# Autodesk Inventor assembly: Plataforma_giratoria_4p
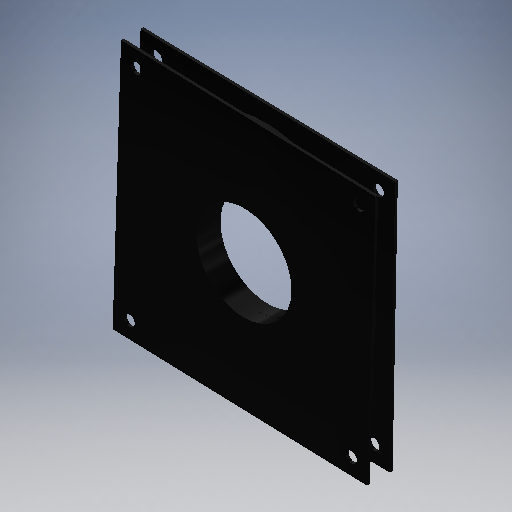
[picture p0: Inventor's stored thumbnail of the model, 512x512]
Saved by Autodesk Inventor 2025.2 (Build 292293000, 293)
## iProperties
Created: 2025-04-27
Part Number: Plataforma_giratoria_4p
Document SubType Name: Assembly
Designer: Tiago
Author: Tiago
## Documents named in this file (2)
- C:\Users\Tiago\Documents\Inventor\Exp. Braço v1\Plataforma_giratoria_4p.iam
- C:\Users\Tiago\Documents\Inventor\Exp. Braço v1\plataforma_giratória_94L)4polegadas).ipt
## Components (2 placed, 1 different names)
1. plataforma_giratória_94L)4polegadas):1 — Mate:1, Mate:2, Flush:1
2. plataforma_giratória_94L)4polegadas):2 — Mate:1, Mate:2
## Relationships (3: Mate 2, Flush 1)
- Mate:1: plataforma_giratória_94L)4polegadas):1 ↔ plataforma_giratória_94L)4polegadas):2
- Mate:2: plataforma_giratória_94L)4polegadas):1 ↔ plataforma_giratória_94L)4polegadas):2
- Flush:1: plataforma_giratória_94L)4polegadas):1
